# Autodesk Inventor assembly: shim_subassembly
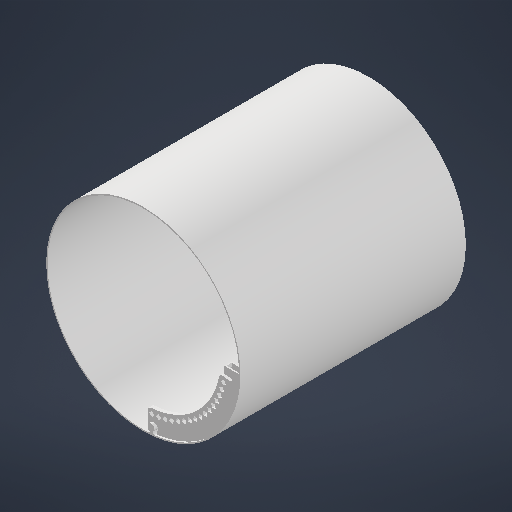
[picture p0: Inventor's stored thumbnail of the model, 512x512]
Saved by Autodesk Inventor 2026.1 (Build 301233020, 233B)
## iProperties
Created: 2025-11-19
Part Number: shim_subassembly
Document SubType Name: Assembly
Designer: Carla Fernandez
Author: Carla Fernandez
## Documents named in this file (3)
- C:\Users\Carla Fernandez\Documents\GitHub\OSII_MINI_V2\CAD MODELS_screw_on\shim_subassembly.iam
- C:\Users\Carla Fernandez\Documents\GitHub\OSII_MINI_V2\CAD MODELS_screw_on\shim_former.ipt
- C:\Users\Carla Fernandez\Documents\GitHub\OSII_MINI_V2\CAD MODELS_screw_on\shim_cartridge.ipt
## Components (2 placed, 2 different names)
1. shim_former:1 — Flush:1, Flush:2, Flush:3, Mate:1, Flush:4
2. shim_cartridge:1 — Mate:1, Flush:4
## Relationships (5: Flush 4, Mate 1)
- Flush:1: shim_former:1
- Flush:2: shim_former:1
- Flush:3: shim_former:1
- Mate:1: shim_former:1 ↔ shim_cartridge:1
- Flush:4 (1.5 mm): shim_former:1 ↔ shim_cartridge:1
